# Autodesk Inventor assembly: controbacion
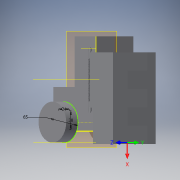
[picture p0: Inventor's stored thumbnail of the model, 180x180]
Saved by Autodesk Inventor 2018 (Build 220112000, 112)
## iProperties
Created: 2019-02-12
Part Number: controbacion
Material: Genérico
Document SubType Name: Assembly
Designer: EDWIN
Author: EDWIN
## Documents named in this file (5)
- C:\Users\EDWIN\Desktop\Inventor\controbacion.iam
- C:\Users\EDWIN\Desktop\Inventor\Pieza1.ipt
- C:\Users\EDWIN\Desktop\Inventor\garra.ipt
- C:\Users\EDWIN\Desktop\Inventor\garra socialista.ipt
- C:\Users\EDWIN\Desktop\Inventor\garra gringa-01.ipt
## Components (4 placed, 4 different names)
1. Pieza1:1 — Coincidencia:1, De rotación:1, De rotación:2, Coincidencia:4
2. garra:1 — Coincidencia:1
3. garra gringa-01:1 — De rotación:1
4. garra socialista:1 — De rotación:2
## Relationships (6: Mate 4, RevoluteJoint 2)
- Coincidencia:1 [Mate]: Pieza1:1 ↔ garra:1
- De rotación:1 [RevoluteJoint]: Pieza1:1 ↔ garra gringa-01:1
- De rotación:2 [RevoluteJoint]: Pieza1:1 ↔ garra socialista:1
- Coincidencia:2 [Mate]
- Coincidencia:3 [Mate]
- Coincidencia:4 [Mate]: Pieza1:1
